# Autodesk Inventor assembly: AssemblyGefreesdBasev2
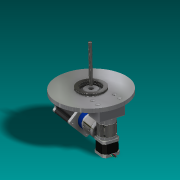
[picture p0: Inventor's stored thumbnail of the model, 180x180]
Saved by Autodesk Inventor 2020.2 (Build 242310000, 310)
## iProperties
Created: 2020-05-18
Part Number: AssemblyGefreesdBasev2
Document SubType Name: Assembly
Designer: Svend
Author: Svend
## Documents named in this file (13)
- C:\Users\Svend\OneDrive\Documents\GitHub\BeerMinder\3D-model\Base (Axis 1)\gefreesd\AssemblyGefreesdBasev2.iam
- C:\Users\Svend\OneDrive\Documents\GitHub\BeerMinder\3D-model\subAssembly\Nema17MetGearbox.iam
- C:\Users\Svend\OneDrive\Documents\GitHub\BeerMinder\3D-model\gearbox\afstandsplaatje.ipt
- C:\Users\Svend\OneDrive\Documents\GitHub\BeerMinder\3D-model\bearings\Ball Bearing 608ZZ.ipt
- C:\Users\Svend\OneDrive\Documents\GitHub\BeerMinder\3D-model\pulleys\GT2 Timing Pulley 20T - 8mm as.ipt
- C:\Users\Svend\OneDrive\Documents\GitHub\BeerMinder\3D-model\pulleys\GT2 Timing Pulley 60T - 8mm as.ipt
- C:\Users\Svend\OneDrive\Documents\GitHub\BeerMinder\3D-model\pulleys\Tandriem20naar60T.ipt
- C:\Users\Svend\OneDrive\Documents\GitHub\BeerMinder\3D-model\Base (Axis 1)\AsBase.ipt
- C:\Users\Svend\OneDrive\Documents\GitHub\BeerMinder\3D-model\subAssembly\Nema23MetGearbox.iam
- C:\Users\Svend\OneDrive\Documents\GitHub\BeerMinder\3D-model\Base (Axis 1)\gefreesd\base bovenkant v2.ipt
- C:\Users\Svend\OneDrive\Documents\GitHub\BeerMinder\3D-model\Base (Axis 1)\gefreesd\onderkant base.ipt
- C:\Users\Svend\OneDrive\Documents\GitHub\BeerMinder\3D-model\bearings\51110 Groefkogellager - 70 mm.iam
- C:\Users\Svend\OneDrive\Documents\GitHub\BeerMinder\3D-model\Base (Axis 1)\gefreesd\hoefijzer.ipt
## Components (12 placed, 12 different names)
1. base bovenkant v2:1 — Mate:20, Mate:7, Flush:5, Mate:46, Flush:7, Flush:8
2. Nema17MetGearbox:1 [sub-assembly] — Mate:20, Mate:52, Mate:56, Mate:58, Mate:59, Flush:6
3. Ball Bearing 608ZZ:1 — Mate:7, Mate:17, Flush:5, Mate:51
4. GT2 Timing Pulley 20T - 8mm as:1 — Mate:52, Mate:53, Mate:54, Flush:6
5. GT2 Timing Pulley 60T - 8mm as:1 — Mate:14, Mate:40, Mate:51, Mate:55
6. Tandriem20naar60T:1 — Mate:14, Mate:53, Mate:54, Mate:55
7. AsBase:1 — Mate:17, Mate:40, Mate:45
8. Nema23MetGearbox:1 [sub-assembly]
9. onderkant base:1
10. 51110 Groefkogellager - 70 mm:1 [sub-assembly] — Mate:45, Mate:46
11. afstandsplaatje:1 — Mate:56, Mate:58, Mate:59
12. hoefijzer:1 — Flush:7, Flush:8
## Relationships (19: Mate 15, Flush 4)
- Mate:20: base bovenkant v2:1 ↔ Nema17MetGearbox:1
- Mate:7: base bovenkant v2:1 ↔ Ball Bearing 608ZZ:1
- Mate:14: GT2 Timing Pulley 60T - 8mm as:1 ↔ Tandriem20naar60T:1
- Mate:17: Ball Bearing 608ZZ:1 ↔ AsBase:1
- Mate:40: GT2 Timing Pulley 60T - 8mm as:1 ↔ AsBase:1
- Flush:5: base bovenkant v2:1 ↔ Ball Bearing 608ZZ:1
- Mate:45: AsBase:1 ↔ 51110 Groefkogellager - 70 mm:1
- Mate:46: base bovenkant v2:1 ↔ 51110 Groefkogellager - 70 mm:1
- Mate:51: Ball Bearing 608ZZ:1 ↔ GT2 Timing Pulley 60T - 8mm as:1
- Mate:52: Nema17MetGearbox:1 ↔ GT2 Timing Pulley 20T - 8mm as:1
- Mate:53 (0.5 mm): GT2 Timing Pulley 20T - 8mm as:1 ↔ Tandriem20naar60T:1
- Mate:54: GT2 Timing Pulley 20T - 8mm as:1 ↔ Tandriem20naar60T:1
- Mate:55 (0.5 mm): GT2 Timing Pulley 60T - 8mm as:1 ↔ Tandriem20naar60T:1
- Mate:56: Nema17MetGearbox:1 ↔ afstandsplaatje:1
- Mate:58: Nema17MetGearbox:1 ↔ afstandsplaatje:1
- Mate:59: Nema17MetGearbox:1 ↔ afstandsplaatje:1
- Flush:6: Nema17MetGearbox:1 ↔ GT2 Timing Pulley 20T - 8mm as:1
- Flush:7: base bovenkant v2:1 ↔ hoefijzer:1
- Flush:8: base bovenkant v2:1 ↔ hoefijzer:1
